# Autodesk Inventor assembly: CNC2
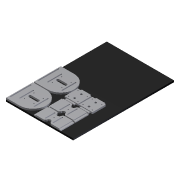
[picture p0: Inventor's stored thumbnail of the model, 180x180]
Saved by Autodesk Inventor 2011 SP1 (Build 150282100, 282)
## iProperties
Created: 2012-12-03
Part Number: CNC2
Document SubType Name: Assembly
Designer: arihon
Author: arihon
## Documents named in this file (5)
- C:\Users\arihon\Dropbox\Inventor\walkPivot\CNC2.iam
- C:\Users\arihon\Dropbox\Inventor\walkPivot\CNC.ipt
- C:\Users\arihon\Dropbox\Inventor\walkPivot\JointB1.ipt
- C:\Users\arihon\Dropbox\Inventor\walkPivot\JointB2.ipt
- C:\Users\arihon\Dropbox\Inventor\walkPivot\JointC0_.ipt
## Components (7 placed, 4 different names)
1. CNC:1 — フラッシュ:1, フラッシュ:2, メイト:1, メイト:2, フラッシュ:3, メイト:4, メイト:5, フラッシュ:4, メイト:7
2. JointB1:1 — フラッシュ:1, メイト:1, フラッシュ:3, メイト:3, 正接:1
3. JointB1:2 — フラッシュ:2, メイト:2, メイト:3
4. JointB2:1 — メイト:5, フラッシュ:4, メイト:6, フラッシュ:5, 正接:1
5. JointB2:2 — メイト:4, メイト:6, フラッシュ:5, フラッシュ:7, メイト:9
6. JointC0_:1 — フラッシュ:6, メイト:7, メイト:8, フラッシュ:8, メイト:9
7. JointC0_:2 — フラッシュ:6, フラッシュ:7, メイト:8, フラッシュ:8
## Relationships (18: Mate 9, Flush 8, Tangent 1)
- フラッシュ:1 [Flush]: CNC:1 ↔ JointB1:1
- フラッシュ:2 [Flush]: CNC:1 ↔ JointB1:2
- メイト:1 [Mate]: CNC:1 ↔ JointB1:1
- メイト:2 [Mate]: CNC:1 ↔ JointB1:2
- フラッシュ:3 [Flush]: CNC:1 ↔ JointB1:1
- メイト:3 [Mate] (3 mm): JointB1:1 ↔ JointB1:2
- メイト:4 [Mate]: CNC:1 ↔ JointB2:2
- メイト:5 [Mate]: CNC:1 ↔ JointB2:1
- フラッシュ:4 [Flush]: CNC:1 ↔ JointB2:1
- メイト:6 [Mate] (3 mm): JointB2:1 ↔ JointB2:2
- フラッシュ:5 [Flush]: JointB2:1 ↔ JointB2:2
- 正接:1 [Tangent] (3 mm): JointB1:1 ↔ JointB2:1
- フラッシュ:6 [Flush]: JointC0_:1 ↔ JointC0_:2
- メイト:7 [Mate]: CNC:1 ↔ JointC0_:1
- フラッシュ:7 [Flush]: JointB2:2 ↔ JointC0_:2
- メイト:8 [Mate] (3 mm): JointC0_:1 ↔ JointC0_:2
- フラッシュ:8 [Flush]: JointC0_:1 ↔ JointC0_:2
- メイト:9 [Mate] (3 mm): JointB2:2 ↔ JointC0_:1
